# Autodesk Inventor assembly: Montagem1
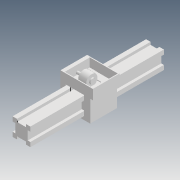
[picture p0: Inventor's stored thumbnail of the model, 180x180]
Saved by Autodesk Inventor 2021 (Build 250183000, 183)
## iProperties
Created: 2020-10-09
Part Number: Montagem1
Document SubType Name: Assembly
Designer: evert
Author: evert
## Documents named in this file (4)
- C:\Users\evert\OneDrive\Área de Trabalho\peca move\Montagem1.iam
- C:\Users\evert\OneDrive\Área de Trabalho\peca move\Peça16.ipt
- C:\Users\evert\OneDrive\Área de Trabalho\peca move\Peça8.ipt
- C:\Users\evert\Downloads\Viga_Projeto_Bosch.ipt
## Components (3 placed, 3 different names)
1. Peça16:1 — Rotativa:1, Conjunto de gaveta:1
2. Peça8:1 — Rotativa:1
3. Viga_Projeto_Bosch:1 — Conjunto de gaveta:1
## Relationships (2: RevoluteJoint 1, TranslationJoint 1)
- Rotativa:1 [RevoluteJoint]: Peça16:1 ↔ Peça8:1
- Conjunto de gaveta:1 [TranslationJoint]: Peça16:1 ↔ Viga_Projeto_Bosch:1
